# Autodesk Inventor assembly: CanSat
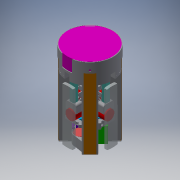
[picture p0: Inventor's stored thumbnail of the model, 180x180]
Saved by Autodesk Inventor 2018 (Build 220112000, 112)
## iProperties
Created: 2018-05-01
Part Number: CanSat
Document SubType Name: Assembly
Designer: suchanek
Author: suchanek
## Documents named in this file (26)
- C:\Users\Suchanek\Programming\CanSat\CanSat2.0\Schematics\Model\CanSat.iam
- C:\Users\Suchanek\Programming\CanSat\CanSat2.0\Schematics\Model\Hull_middle.ipt
- C:\Users\Suchanek\Programming\CanSat\CanSat2.0\Schematics\Model\Circuit.ipt
- C:\Users\Suchanek\Programming\CanSat\CanSat2.0\Schematics\Model\Motor_drivers.ipt
- C:\Users\Suchanek\Programming\CanSat\CanSat2.0\Schematics\Model\Hull_main.ipt
- C:\Users\Suchanek\Programming\CanSat\CanSat2.0\Schematics\Model\Circuit_center.ipt
- C:\Users\Suchanek\Programming\CanSat\CanSat2.0\Schematics\Model\Arm.ipt
- C:\Users\Suchanek\Programming\CanSat\CanSat2.0\Schematics\Model\Motor_holder.ipt
- C:\Users\Suchanek\Programming\CanSat\CanSat2.0\Schematics\Model\Motor.ipt
- C:\Users\Suchanek\Programming\CanSat\CanSat2.0\Schematics\Model\Rotor.ipt
- C:\Users\Suchanek\Programming\CanSat\CanSat2.0\Schematics\Model\Flight_controler.ipt
- C:\Users\Suchanek\Programming\CanSat\CanSat2.0\Schematics\Model\SIM808.ipt
- C:\Users\Suchanek\Programming\CanSat\CanSat2.0\Schematics\Model\Batt_pillar.ipt
- C:\Users\Suchanek\Programming\CanSat\CanSat2.0\Schematics\Model\Servo.ipt
- C:\Users\Suchanek\Programming\CanSat\CanSat2.0\Schematics\Model\Servo_bit.ipt
- C:\Users\Suchanek\Programming\CanSat\CanSat2.0\Schematics\Model\Spring.ipt
- C:\Users\Suchanek\Programming\CanSat\CanSat2.0\Schematics\Model\Scraper.ipt
- C:\Users\Suchanek\Programming\CanSat\CanSat2.0\Schematics\Model\Camera.ipt
- C:\Users\Suchanek\Programming\CanSat\CanSat2.0\Schematics\Model\Cam_SD_base.ipt
- C:\Users\Suchanek\Programming\CanSat\CanSat2.0\Schematics\Model\Cam_SD_chip.ipt
- C:\Users\Suchanek\Programming\CanSat\CanSat2.0\Schematics\Model\Hull_batt_pillar1.ipt
- C:\Users\Suchanek\Programming\CanSat\CanSat2.0\Schematics\Model\Hull_batt_pillar3.ipt
- C:\Users\Suchanek\Programming\CanSat\CanSat2.0\Schematics\Model\Hull_batt_pillar2.ipt
- C:\Users\Suchanek\Programming\CanSat\CanSat2.0\Schematics\Model\Hull_batt_pillar4.ipt
- C:\Users\Suchanek\Programming\CanSat\CanSat2.0\Schematics\Model\gamma.ipt
- C:\Users\Suchanek\Programming\CanSat\CanSat2.0\Schematics\Model\Cam_antenna.ipt
## Components (40 placed, 25 different names)
1. Hull_middle:1 — Rotational:3, Flush:2, Mate:9
2. Circuit:1 — Rotational:21
3. Motor_drivers:1 — Flush:1, Angle:4, Cylindrical:1, Mate:1
4. Hull_main:1 — Rotational:3, Flush:1, Angle:4, Cylindrical:1, Mate:3, Mate:6, Tangent:1, Rotační:15, Rotational:18, Mate:21, Rotational:19, Mate:22, Rotational:20, Mate:23, Rotational:21, Rotational:22, Mate:24
5. Circuit_center:1 — Flush:2, Mate:9, Tangent:1, Proti sobě:10, Proti sobě:11
6. Flight_controler:1 — Mate:1, Mate:2, Flush:4, Symmetry:1
7. SIM808:1 — Mate:2, Flush:4, Symmetry:1
8. Servo:1 — Rotational:6, Proti sobě:16, Stejný směr:13, Mate:25, Angle:14
9. Servo_bit:1 — Rotational:6, Rigid:3, Angle:11
10. Spring:1 — Rigid:3, Rotational:7
11. Scraper:1 — Rotational:7, Angle:11
12. Camera:1 — Rotational:17, Angle:14
13. Cam_SD_base:1 — Mate:26, Flush:15, Mate:27
14. Cam_SD_chip:1 — Rigid:4
15. Hull_batt_pillar1:1 — Proti sobě:18, Rotational:19, Mate:22
16. Hull_batt_pillar3:1 — Proti sobě:12, Proti sobě:15, Flush:14, Mate:20, Rotational:17, Rotational:20, Mate:23, Rotational:23, Mate:25
17. Hull_batt_pillar2:1 — Rotational:22, Mate:24, Rigid:4, Mate:26, Flush:15, Mate:27
18. Hull_batt_pillar4:1 — Proti sobě:16, Stejný směr:13, Proti sobě:17, Rotational:18, Mate:21
19. gamma:1 — Proti sobě:10, Proti sobě:11, Proti sobě:12, Proti sobě:19
20. Cam_antenna:1 — Flush:14, Rotational:23
21. Arm:1 — Rigid:1, Rotační:15
22. Motor_holder:1 — Rigid:1, Rigid:2
23. Motor:1 — Rigid:2, Rotational:5
24. Rotor:1 — Rotational:5
25. Arm:2
26. Motor_holder:2
27. Motor:2
28. Rotor:2
29. Arm:3
30. Motor_holder:3
31. Motor:3
32. Rotor:3
33. Arm:4
34. Motor_holder:4
35. Motor:4
36. Rotor:4
37. Batt_pillar:1 — Mate:6
38. Batt_pillar:2
39. Batt_pillar:3
40. Batt_pillar:4
## Component patterns: (4 elements, first: Arm:1 + Motor_holder:1 + Motor:1 + Rotor:1), (4 elements, first: Batt_pillar:1)
## Relationships (51: Mate 23, RevoluteJoint 12, Flush 6, WeldJoint 4, Angle 3, CylindricalJoint 1, Symmetry 1, Tangent 1)
- Rotational:3 [RevoluteJoint]: Hull_middle:1 ↔ Hull_main:1
- Flush:1 (12 mm): Motor_drivers:1 ↔ Hull_main:1
- Angle:4 (0 deg): Motor_drivers:1 ↔ Hull_main:1
- Cylindrical:1: Motor_drivers:1 ↔ Hull_main:1
- Flush:2 (3 mm): Hull_middle:1 ↔ Circuit_center:1
- Rigid:1 [WeldJoint]: Arm:1 ↔ Motor_holder:1
- Rigid:2 [WeldJoint]: Motor_holder:1 ↔ Motor:1
- Rotational:5 [RevoluteJoint]: Motor:1 ↔ Rotor:1
- Mate:1 (5 mm): Motor_drivers:1 ↔ Flight_controler:1
- Mate:2 (2 mm): Flight_controler:1 ↔ SIM808:1
- Mate:3: Hull_main:1
- Mate:4
- Mate:5
- Flush:4 (-0.5 mm): Flight_controler:1 ↔ SIM808:1
- Mate:6: Hull_main:1 ↔ Batt_pillar:1
- Symmetry:1: Flight_controler:1 ↔ SIM808:1
- Rotational:6 [RevoluteJoint]: Servo:1 ↔ Servo_bit:1
- Rigid:3 [WeldJoint]: Servo_bit:1 ↔ Spring:1
- Rotational:7 [RevoluteJoint]: Spring:1 ↔ Scraper:1
- Angle:11 (0 deg): Servo_bit:1 ↔ Scraper:1
- Mate:9 (0.245 mm): Hull_middle:1 ↔ Circuit_center:1
- Tangent:1 (-16.4 mm): Hull_main:1 ↔ Circuit_center:1
- Proti sobě:10 [Mate] (-28 mm): Circuit_center:1 ↔ gamma:1
- Proti sobě:11 [Mate]: Circuit_center:1 ↔ gamma:1
- Proti sobě:12 [Mate] (3.163 mm): Hull_batt_pillar3:1 ↔ gamma:1
- Proti sobě:15 [Mate]: Hull_batt_pillar3:1
- Proti sobě:16 [Mate]: Servo:1 ↔ Hull_batt_pillar4:1
- Stejný směr:13 [Flush]: Servo:1 ↔ Hull_batt_pillar4:1
- Rotační:15 [RevoluteJoint]: Hull_main:1 ↔ Arm:1
- Proti sobě:17 [Mate]: Hull_batt_pillar4:1
- Proti sobě:18 [Mate]: Hull_batt_pillar1:1
- Proti sobě:19 [Mate]: gamma:1
- Flush:14: Hull_batt_pillar3:1 ↔ Cam_antenna:1
- Mate:20: Hull_batt_pillar3:1
- Rotational:17 [RevoluteJoint]: Camera:1 ↔ Hull_batt_pillar3:1
- Rotational:18 [RevoluteJoint]: Hull_main:1 ↔ Hull_batt_pillar4:1
- Mate:21: Hull_main:1 ↔ Hull_batt_pillar4:1
- Rotational:19 [RevoluteJoint]: Hull_main:1 ↔ Hull_batt_pillar1:1
- Mate:22: Hull_main:1 ↔ Hull_batt_pillar1:1
- Rotational:20 [RevoluteJoint]: Hull_main:1 ↔ Hull_batt_pillar3:1
- Mate:23: Hull_main:1 ↔ Hull_batt_pillar3:1
- Rotational:21 [RevoluteJoint]: Circuit:1 ↔ Hull_main:1
- Rotational:22 [RevoluteJoint]: Hull_main:1 ↔ Hull_batt_pillar2:1
- Mate:24: Hull_main:1 ↔ Hull_batt_pillar2:1
- Rotational:23 [RevoluteJoint]: Hull_batt_pillar3:1 ↔ Cam_antenna:1
- Mate:25 (0.25 mm): Servo:1 ↔ Hull_batt_pillar3:1
- Angle:14 (0 deg): Servo:1 ↔ Camera:1
- Rigid:4 [WeldJoint] (0.1 mm): Cam_SD_chip:1 ↔ Hull_batt_pillar2:1
- Mate:26: Cam_SD_base:1 ↔ Hull_batt_pillar2:1
- Flush:15 (1 mm): Cam_SD_base:1 ↔ Hull_batt_pillar2:1
- Mate:27: Cam_SD_base:1 ↔ Hull_batt_pillar2:1
